# Autodesk Inventor assembly: MGN-12H
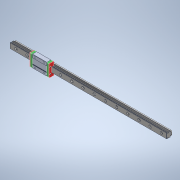
[picture p0: Inventor's stored thumbnail of the model, 180x180]
Saved by Autodesk Inventor 2022 (Build 260153000, 153)
## iProperties
Created: 2021-10-05
Part Number: MGN-12H
Document SubType Name: Assembly
Designer: nicol
Author: nicol
## Documents named in this file (8)
- Y:\Projects\Bibble0\Hardware\MGN-12H\MGN-12H.iam
- Y:\Projects\Bibble0\Hardware\MGN-12H\Button M3x8.ipt
- Y:\Projects\Bibble0\Hardware\MGN-12H\Green End Cap.ipt
- Y:\Projects\Bibble0\Hardware\MGN-12H\Main Block.ipt
- Y:\Projects\Bibble0\Hardware\MGN-12H\Red End Cap.ipt
- Y:\Projects\Bibble0\Hardware\MGN-12H\Rail 400mm.ipt
- Y:\Projects\Bibble0\Sheet Metal\Linear Rail Screw Plate.ipt
- Y:\Projects\Bibble0\Hardware\M3 x 8 mm SHCS.ipt
## Components (25 placed, 7 different names)
1. Button M3x8:1 — Insert:12
2. Green End Cap:1 — Insert:1, Insert:2, Insert:3, Insert:4
3. Main Block:1 — Insert:1, Insert:2, Insert:5, Insert:6, Mate:1, Mate:2
4. Green End Cap:2 — Insert:5, Insert:6, Insert:7, Insert:8
5. Red End Cap:1 — Insert:3, Insert:4, Insert:11, Insert:12
6. Red End Cap:2 — Insert:7, Insert:8, Insert:9, Insert:10, Flush:1
7. Button M3x8:2 — Insert:9
8. Button M3x8:3 — Insert:10
9. Button M3x8:4 — Insert:11
10. Rail 400mm:1 — Mate:1, Mate:2, Flush:1, Insert:13, Mate:3, Insert:14
11. Linear Rail Screw Plate:1 — Insert:13, Mate:3
12. M3 x 8 mm SHCS:1 — Insert:14
13. M3 x 8 mm SHCS:2
14. M3 x 8 mm SHCS:3
15. M3 x 8 mm SHCS:4
16. M3 x 8 mm SHCS:5
17. M3 x 8 mm SHCS:6
18. M3 x 8 mm SHCS:7
19. M3 x 8 mm SHCS:8
20. M3 x 8 mm SHCS:9
21. M3 x 8 mm SHCS:10
22. M3 x 8 mm SHCS:11
23. M3 x 8 mm SHCS:12
24. M3 x 8 mm SHCS:13
25. M3 x 8 mm SHCS:14
## Component patterns: (14 elements, first: M3 x 8 mm SHCS:1)
## Relationships (18: Insert 14, Mate 3, Flush 1)
- Insert:1: Green End Cap:1 ↔ Main Block:1
- Insert:2: Green End Cap:1 ↔ Main Block:1
- Insert:3: Green End Cap:1 ↔ Red End Cap:1
- Insert:4: Green End Cap:1 ↔ Red End Cap:1
- Insert:5: Main Block:1 ↔ Green End Cap:2
- Insert:6: Main Block:1 ↔ Green End Cap:2
- Insert:7: Green End Cap:2 ↔ Red End Cap:2
- Insert:8: Green End Cap:2 ↔ Red End Cap:2
- Insert:9: Red End Cap:2 ↔ Button M3x8:2
- Insert:10: Red End Cap:2 ↔ Button M3x8:3
- Insert:11: Red End Cap:1 ↔ Button M3x8:4
- Insert:12: Button M3x8:1 ↔ Red End Cap:1
- Mate:1: Main Block:1 ↔ Rail 400mm:1
- Mate:2: Main Block:1 ↔ Rail 400mm:1
- Flush:1: Red End Cap:2 ↔ Rail 400mm:1
- Insert:13 (1.5 mm): Rail 400mm:1 ↔ Linear Rail Screw Plate:1
- Mate:3: Rail 400mm:1 ↔ Linear Rail Screw Plate:1
- Insert:14: Rail 400mm:1 ↔ M3 x 8 mm SHCS:1
